# Autodesk Inventor assembly: FinAssNut_Bolt
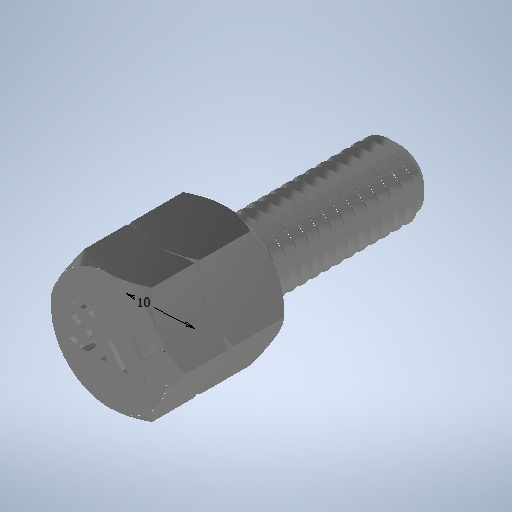
[picture p0: Inventor's stored thumbnail of the model, 512x512]
Saved by Autodesk Inventor 2025.2 (Build 292293000, 293)
## iProperties
Created: 2025-05-10
Part Number: FinAssNut_Bolt
Document SubType Name: Assembly
Designer: spars
Author: spars
## Documents named in this file (3)
- C:\Users\spars\OneDrive\Desktop\2nd Semester\Inventor\CAD@Start\FinAssNut_Bolt.iam
- C:\Users\spars\OneDrive\Desktop\2nd Semester\Inventor\CAD@Start\cad@18.ipt
- C:\Users\spars\OneDrive\Desktop\2nd Semester\Inventor\CAD@Start\cad@19.ipt
## Components (2 placed, 2 different names)
1. cad@18:1 — Mate:1, Flush:1, Angle:1
2. cad@19:1 — Mate:1, Flush:1, Angle:1
## Relationships (3: Mate 1, Flush 1, Angle 1)
- Mate:1: cad@18:1 ↔ cad@19:1
- Flush:1: cad@18:1 ↔ cad@19:1
- Angle:1 (0 deg): cad@18:1 ↔ cad@19:1
